# Autodesk Inventor assembly: Arduino_Oktagon
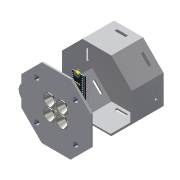
[picture p0: Inventor's stored thumbnail of the model, 180x180]
Saved by Autodesk Inventor 2018.2 (Build 222227000, 227)
## iProperties
Company: Fraunhofer ILT
Created: 2018-10-01
Part Number: Arduino_Oktagon
Material: geeigneten Werkstoff auswählen !
Document SubType Name: Assembly
Designer: N.Grubert
Title: =Description
Author: N.Grubert
## Documents named in this file (5)
- C:\Users\GRUBERT\Documents\COSIMA-Laserstar\CAD\Arduino_Oktagon.iam
- C:\Users\GRUBERT\Documents\COSIMA-Laserstar\CAD\Oktagon.ipt
- C:\Users\GRUBERT\Documents\COSIMA-Laserstar\CAD\DeckelParabol.iam
- C:\Users\GRUBERT\Downloads\arduino-micro-1.snapshot.2\ARDUINO MICRO.iam
- C:\Users\GRUBERT\Documents\COSIMA-Laserstar\CAD\Kühlkörper.ipt
## Components (4 placed, 4 different names)
1. Oktagon:1 — Passend:1, Passend:2, Passend:3, Passend:4, Fluchtend:1, Fluchtend:2, Passend:5
2. DeckelParabol:1 [sub-assembly] — Fluchtend:1, Fluchtend:2, Passend:5, Passend:6, Winkel:1
3. ARDUINO MICRO:1 [sub-assembly] — Winkel:1, Passend:7
4. Kühlkörper:1 — Passend:6, Passend:7
## Relationships (10: Mate 7, Flush 2, Angle 1)
- Passend:1 [Mate]: Oktagon:1
- Passend:2 [Mate]: Oktagon:1
- Passend:3 [Mate]: Oktagon:1
- Passend:4 [Mate]: Oktagon:1
- Fluchtend:1 [Flush]: Oktagon:1 ↔ DeckelParabol:1
- Fluchtend:2 [Flush]: Oktagon:1 ↔ DeckelParabol:1
- Passend:5 [Mate]: Oktagon:1 ↔ DeckelParabol:1
- Passend:6 [Mate]: DeckelParabol:1 ↔ Kühlkörper:1
- Winkel:1 [Angle] (0 deg): DeckelParabol:1 ↔ ARDUINO MICRO:1
- Passend:7 [Mate] (5 mm): ARDUINO MICRO:1 ↔ Kühlkörper:1
